# Autodesk Inventor assembly: Dog Feeder
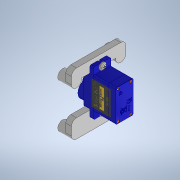
[picture p0: Inventor's stored thumbnail of the model, 180x180]
Saved by Autodesk Inventor 2020.1 (Build 241239000, 239)
## iProperties
Created: 2019-11-16
Part Number: Dog Feeder
Document SubType Name: Assembly
Designer: Daniel
Author: Daniel
## Documents named in this file (7)
- F:\Proyectos\Dog Feeder\Solido\Dog Feeder.iam
- F:\Proyectos\Dog Feeder\Solido\Dosificador.ipt
- F:\Proyectos\Dog Feeder\Solido\Soporte.ipt
- F:\Proyectos\Dog Feeder\Solido\Pata.ipt
- F:\Proyectos\Dog Feeder\Solido\Exagono.ipt
- F:\Proyectos\Dog Feeder\Solido\Soporte_Servo.ipt
- F:\Proyectos\Dog Feeder\Solido\Servo SG90\SG90 - Micro Servo 9g - Tower Pro.iam
## Components (7 placed, 6 different names)
1. Dosificador:1 — Rotational:1, Flush:4, Flush:6
2. Soporte:1 — Flush:1, Flush:2, Rotational:1, Flush:3, Mate:4, Mate:6, Mate:7, Flush:7
3. Pata:1 — Flush:3
4. Pata:2 — Mate:4, Mate:6, Mate:7
5. Exagono:1 — Flush:4, Flush:6, Insert:1, Mate:8
6. Soporte_Servo:1 — Flush:7
7. SG90 - Micro Servo 9g - Tower Pro:1 [sub-assembly] — Insert:1, Mate:8, Flush:8
## Relationships (13: Flush 7, Mate 4, RevoluteJoint 1, Insert 1)
- Flush:1: Soporte:1
- Flush:2: Soporte:1
- Rotational:1 [RevoluteJoint]: Dosificador:1 ↔ Soporte:1
- Flush:3: Soporte:1 ↔ Pata:1
- Mate:4: Soporte:1 ↔ Pata:2
- Mate:6: Soporte:1 ↔ Pata:2
- Flush:4: Dosificador:1 ↔ Exagono:1
- Flush:6: Dosificador:1 ↔ Exagono:1
- Mate:7: Soporte:1 ↔ Pata:2
- Flush:7: Soporte:1 ↔ Soporte_Servo:1
- Insert:1: Exagono:1 ↔ SG90 - Micro Servo 9g - Tower Pro:1
- Mate:8: Exagono:1 ↔ SG90 - Micro Servo 9g - Tower Pro:1
- Flush:8 (7.08 mm): SG90 - Micro Servo 9g - Tower Pro:1
